# Autodesk Inventor assembly: Head
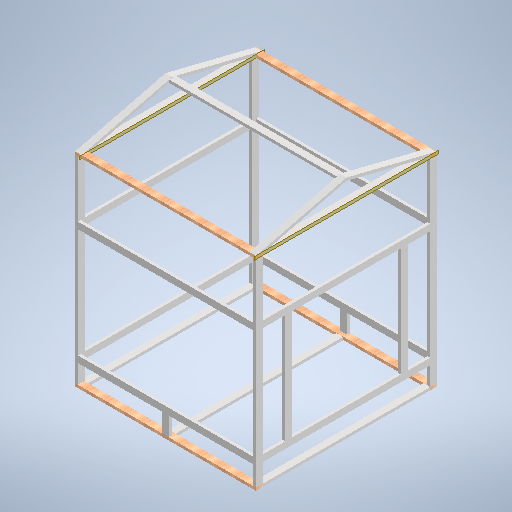
[picture p0: Inventor's stored thumbnail of the model, 512x512]
Saved by Autodesk Inventor 2025 (Build 290162000, 162)
## iProperties
Created: 2024-09-18
Part Number: Head
Document SubType Name: Assembly
Designer: localadmin
Author: localadmin
## Documents named in this file (9)
- C:\Users\localadmin\Documents\USCTigerBurn24\Head.iam
- C:\Users\localadmin\Documents\USCTigerBurn24\Standard Timber\2x4x96.ipt
- C:\Users\localadmin\Documents\USCTigerBurn24\Standard Timber\7'5''x2x4Correct.ipt
- C:\Users\localadmin\Documents\USCTigerBurn24\Standard Timber\10'x2x4.ipt
- C:\Users\localadmin\Documents\USCTigerBurn24\Standard Timber\top head slant.ipt
- C:\Users\localadmin\Documents\USCTigerBurn24\Standard Timber\top head slant_MIR.ipt
- C:\Users\localadmin\Documents\USCTigerBurn24\Standard Timber\7'9''x2x4.ipt
- C:\Users\localadmin\Documents\USCTigerBurn24\Standard Timber\10''x2x4.ipt
- C:\Users\localadmin\Documents\USCTigerBurn24\Standard Timber\4'10''x2x4.ipt
## Components (30 placed, 8 different names)
1. 2x4x96:1 — Flush:1, Mate:1, Flush:2, Mate:2, Flush:3, Flush:4, Mate:3, Flush:7, Flush:8, Mate:5, Flush:11, Flush:12, Mate:7, Flush:15, Flush:16, Mate:12, Flush:49, Mate:33
2. 2x4x96:2 — Flush:1, Mate:1, Flush:2, Flush:5, Flush:6, Mate:4, Flush:9, Flush:10, Mate:6, Flush:13, Flush:14, Flush:47
3. 7'5''x2x4Correct:1 — Mate:2, Flush:3, Flush:4, Flush:5, Flush:6, Flush:27, Mate:13
4. 7'5''x2x4Correct:2 — Mate:3, Flush:7, Flush:8
5. 10'x2x4:1 — Mate:4, Flush:9, Flush:10, Mate:11, Mate:14, Flush:28, Mate:16, Flush:29, Mate:24, Flush:37, Mate:34
6. 10'x2x4:2 — Mate:5, Flush:11, Flush:12, Flush:25, Flush:26, Mate:37
7. 10'x2x4:3 — Mate:6, Flush:13, Flush:14, Flush:35, Mate:23, Mate:25
8. 10'x2x4:4 — Mate:7, Flush:15, Flush:16, Mate:26, Flush:39, Flush:41, Mate:27, Mate:30, Flush:43, Mate:31, Flush:45
9. 2x4x96:3 — Flush:25, Mate:21, Mate:22, Flush:34
10. 2x4x96:4 — Mate:11, Mate:17, Mate:18, Flush:32
11. 7'5''x2x4Correct:3 — Flush:26, Flush:30, Flush:31
12. 7'5''x2x4Correct:4
13. 7'5''x2x4Correct:5 — Mate:12, Flush:27, Flush:48, Flush:50
14. 7'5''x2x4Correct:6 — Mate:13, Mate:14, Flush:28, Mate:15, Flush:36, Flush:42, Flush:51
15. 7'5''x2x4Correct:7 — Mate:15, Mate:16, Flush:29, Flush:38, Flush:40, Mate:35, Mate:36, Flush:52
16. top head slant:1 — Flush:30, Flush:31, Mate:19, Mate:29
17. top head slant_MIR:1 — Mate:17, Mate:18, Flush:32, Mate:19, Mate:28
18. top head slant:2 — Mate:20, Flush:33, Mate:21, Mate:22, Flush:34
19. top head slant_MIR:2 — Mate:20, Flush:33
20. 7'9''x2x4:1 — Flush:35, Mate:23, Flush:36, Mate:32
21. 7'9''x2x4:2 — Mate:24, Mate:25, Flush:37, Flush:38
22. 7'9''x2x4:3 — Mate:26, Flush:39, Flush:40, Flush:46
23. 7'9''x2x4:4 — Flush:41, Mate:27, Flush:42, Flush:44
24. 7'5''x2x4Correct:8 — Mate:28, Mate:29
25. 7'5''x2x4Correct:9 — Mate:30, Flush:43, Flush:44
26. 7'5''x2x4Correct:10 — Mate:31, Flush:45, Flush:46
27. 10''x2x4:1 — Flush:47, Mate:32, Flush:48
28. 10''x2x4:2 — Flush:49, Mate:33, Flush:50
29. 4'10''x2x4:2 — Mate:34, Mate:35, Flush:51
30. 4'10''x2x4:3 — Mate:36, Mate:37, Flush:52
## Relationships (89: Flush 52, Mate 37)
- Flush:1: 2x4x96:1 ↔ 2x4x96:2
- Mate:1 (2260.6 mm): 2x4x96:1 ↔ 2x4x96:2
- Flush:2: 2x4x96:1 ↔ 2x4x96:2
- Mate:2: 2x4x96:1 ↔ 7'5''x2x4Correct:1
- Flush:3: 2x4x96:1 ↔ 7'5''x2x4Correct:1
- Flush:4: 2x4x96:1 ↔ 7'5''x2x4Correct:1
- Flush:5: 2x4x96:2 ↔ 7'5''x2x4Correct:1
- Flush:6: 2x4x96:2 ↔ 7'5''x2x4Correct:1
- Mate:3: 2x4x96:1 ↔ 7'5''x2x4Correct:2
- Flush:7: 2x4x96:1 ↔ 7'5''x2x4Correct:2
- Flush:8: 2x4x96:1 ↔ 7'5''x2x4Correct:2
- Mate:4: 2x4x96:2 ↔ 10'x2x4:1
- Flush:9: 2x4x96:2 ↔ 10'x2x4:1
- Flush:10: 2x4x96:2 ↔ 10'x2x4:1
- Mate:5: 2x4x96:1 ↔ 10'x2x4:2
- Flush:11: 2x4x96:1 ↔ 10'x2x4:2
- Flush:12: 2x4x96:1 ↔ 10'x2x4:2
- Mate:6: 2x4x96:2 ↔ 10'x2x4:3
- Flush:13: 2x4x96:2 ↔ 10'x2x4:3
- Flush:14: 2x4x96:2 ↔ 10'x2x4:3
- Mate:7: 2x4x96:1 ↔ 10'x2x4:4
- Flush:15: 2x4x96:1 ↔ 10'x2x4:4
- Flush:16: 2x4x96:1 ↔ 10'x2x4:4
- [Flush]: 2x4x96:3 ↔ 2x4x96:4
- [Mate] (2260.6 mm): 2x4x96:3 ↔ 2x4x96:4
- [Flush]: 2x4x96:3 ↔ 2x4x96:4
- [Mate]: 2x4x96:3 ↔ 7'5''x2x4Correct:3
- [Flush]: 2x4x96:3 ↔ 7'5''x2x4Correct:3
- [Flush]: 2x4x96:3 ↔ 7'5''x2x4Correct:3
- [Flush]: 2x4x96:4 ↔ 7'5''x2x4Correct:3
- [Flush]: 2x4x96:4 ↔ 7'5''x2x4Correct:3
- [Mate]: 2x4x96:3 ↔ 7'5''x2x4Correct:4
- [Flush]: 2x4x96:3 ↔ 7'5''x2x4Correct:4
- [Flush]: 2x4x96:3 ↔ 7'5''x2x4Correct:4
- Mate:11: 10'x2x4:1 ↔ 2x4x96:4
- Flush:25: 10'x2x4:2 ↔ 2x4x96:3
- Flush:26: 10'x2x4:2 ↔ 7'5''x2x4Correct:3
- Mate:12: 2x4x96:1 ↔ 7'5''x2x4Correct:5
- Flush:27 (1174.75 mm): 7'5''x2x4Correct:1 ↔ 7'5''x2x4Correct:5
- Mate:13 (254 mm): 7'5''x2x4Correct:1 ↔ 7'5''x2x4Correct:6
- Mate:14: 10'x2x4:1 ↔ 7'5''x2x4Correct:6
- Flush:28: 10'x2x4:1 ↔ 7'5''x2x4Correct:6
- Mate:15 (1473.2 mm): 7'5''x2x4Correct:6 ↔ 7'5''x2x4Correct:7
- Mate:16: 10'x2x4:1 ↔ 7'5''x2x4Correct:7
- Flush:29: 10'x2x4:1 ↔ 7'5''x2x4Correct:7
- Flush:30: 7'5''x2x4Correct:3 ↔ top head slant:1
- Flush:31: 7'5''x2x4Correct:3 ↔ top head slant:1
- Mate:17: 2x4x96:4 ↔ top head slant_MIR:1
- Mate:18: 2x4x96:4 ↔ top head slant_MIR:1
- Flush:32: 2x4x96:4 ↔ top head slant_MIR:1
- Mate:19: top head slant:1 ↔ top head slant_MIR:1
- Mate:20: top head slant:2 ↔ top head slant_MIR:2
- Flush:33: top head slant:2 ↔ top head slant_MIR:2
- Mate:21: 2x4x96:3 ↔ top head slant:2
- Mate:22: 2x4x96:3 ↔ top head slant:2
- Flush:34: 2x4x96:3 ↔ top head slant:2
- Flush:35: 10'x2x4:3 ↔ 7'9''x2x4:1
- Mate:23: 10'x2x4:3 ↔ 7'9''x2x4:1
- Flush:36: 7'5''x2x4Correct:6 ↔ 7'9''x2x4:1
- Mate:24: 10'x2x4:1 ↔ 7'9''x2x4:2
- Mate:25: 10'x2x4:3 ↔ 7'9''x2x4:2
- Flush:37: 10'x2x4:1 ↔ 7'9''x2x4:2
- Flush:38: 7'5''x2x4Correct:7 ↔ 7'9''x2x4:2
- Mate:26: 10'x2x4:4 ↔ 7'9''x2x4:3
- Flush:39: 10'x2x4:4 ↔ 7'9''x2x4:3
- Flush:40: 7'5''x2x4Correct:7 ↔ 7'9''x2x4:3
- Flush:41: 10'x2x4:4 ↔ 7'9''x2x4:4
- Mate:27: 10'x2x4:4 ↔ 7'9''x2x4:4
- Flush:42: 7'5''x2x4Correct:6 ↔ 7'9''x2x4:4
- Mate:28: top head slant_MIR:1 ↔ 7'5''x2x4Correct:8
- Mate:29 (44.45 mm): top head slant:1 ↔ 7'5''x2x4Correct:8
- Mate:30: 10'x2x4:4 ↔ 7'5''x2x4Correct:9
- Flush:43: 10'x2x4:4 ↔ 7'5''x2x4Correct:9
- Flush:44: 7'9''x2x4:4 ↔ 7'5''x2x4Correct:9
- Mate:31: 10'x2x4:4 ↔ 7'5''x2x4Correct:10
- Flush:45: 10'x2x4:4 ↔ 7'5''x2x4Correct:10
- Flush:46: 7'9''x2x4:3 ↔ 7'5''x2x4Correct:10
- Flush:47: 2x4x96:2 ↔ 10''x2x4:1
- Mate:32: 7'9''x2x4:1 ↔ 10''x2x4:1
- Flush:48: 7'5''x2x4Correct:5 ↔ 10''x2x4:1
- Flush:49: 2x4x96:1 ↔ 10''x2x4:2
- Mate:33: 2x4x96:1 ↔ 10''x2x4:2
- Flush:50: 7'5''x2x4Correct:5 ↔ 10''x2x4:2
- Mate:34 (304.8 mm): 10'x2x4:1 ↔ 4'10''x2x4:2
- Mate:35: 7'5''x2x4Correct:7 ↔ 4'10''x2x4:2
- Flush:51: 7'5''x2x4Correct:6 ↔ 4'10''x2x4:2
- Mate:36: 7'5''x2x4Correct:7 ↔ 4'10''x2x4:3
- Mate:37 (304.8 mm): 10'x2x4:2 ↔ 4'10''x2x4:3
- Flush:52: 7'5''x2x4Correct:7 ↔ 4'10''x2x4:3
## Named parameters: d39_d16 = 0 mm, d40_d17 = 2260.6 mm, d41_d18 = 0 mm, d42_d19 = 0 mm, d43_d20 = 0 mm, d44_d21 = 0 mm, d45_d22 = 0 mm, d46_d23 = 0 mm, d47_d24 = 0 mm, d48_d25 = 0 mm, d49_d26 = 0 mm
